# Autodesk Inventor assembly: CrossBot
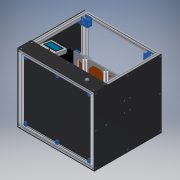
[picture p0: Inventor's stored thumbnail of the model, 180x180]
Saved by Autodesk Inventor 2016 (Build 200138000, 138)
## iProperties
Created: 2014-08-14
Part Number: CrossBot
Document SubType Name: Assembly
Designer: t_clevj
Mass: 16815.8 g
Surface Area: 53062.5 cm^2
Volume: 10946.1 cm^3
Density: 1.53623 g/cm^3
Author: t_clevj
## Documents named in this file (26)
- C:\Users\Jack\ownCloud\Projects\CrossBot\InventorModel\CrossBot.iam
- C:\Users\Jack\ownCloud\Projects\CrossBot\InventorModel\Frame\Frame.iam
- C:\Users\Jack\ownCloud\Projects\CrossBot\InventorModel\Hardware\Shaft\Shaft8\YShaft.ipt
- C:\Users\Jack\ownCloud\Projects\CrossBot\InventorModel\YAxis\YAxisMotorLeft.iam
- C:\Users\Jack\ownCloud\Projects\CrossBot\InventorModel\YAxis\YAxisIdlerLeft.iam
- C:\Users\Jack\ownCloud\Projects\CrossBot\InventorModel\YAxis\YAxisMotorRight.iam
- C:\Users\Jack\ownCloud\Projects\CrossBot\InventorModel\XAxis\XEndLeft.iam
- C:\Users\Jack\ownCloud\Projects\CrossBot\InventorModel\YAxis\YAxisIdlerRight.iam
- C:\Users\Jack\ownCloud\Projects\CrossBot\InventorModel\XAxis\XEndRight.iam
- C:\Users\Jack\ownCloud\Projects\CrossBot\InventorModel\Hardware\Shaft\Shaft8\XShaft.ipt
- C:\Users\Jack\ownCloud\Projects\CrossBot\InventorModel\Hardware\Shaft\Shaft10\ZAxisShaft.ipt
- C:\Users\Jack\ownCloud\Projects\CrossBot\InventorModel\Enclosure\SpoolFilamentToyBuilderLabs.ipt
- C:\Users\Jack\ownCloud\Projects\CrossBot\InventorModel\XAxis\XCarriage.iam
- C:\Users\Jack\ownCloud\Projects\CrossBot\InventorModel\Electronics\PSUUltibots.ipt
- C:\Users\Jack\ownCloud\Projects\CrossBot\InventorModel\ZAxis\ZAxisBed.iam
- C:\Users\Jack\ownCloud\Projects\CrossBot\InventorModel\ZAxis\ZAxisRodClamp.iam
- C:\Users\Jack\ownCloud\Projects\CrossBot\InventorModel\ZAxis\ZDrive.iam
- C:\Users\Jack\ownCloud\Projects\CrossBot\InventorModel\Electronics\KeySwitch\KeySwitch.iam
- C:\Users\Jack\ownCloud\Projects\CrossBot\InventorModel\ZAxis\ZEndstop.iam
- C:\Users\Jack\ownCloud\Projects\CrossBot\InventorModel\Electronics\Ports\PowerSocket.ipt
- C:\Users\Jack\ownCloud\Projects\CrossBot\InventorModel\Hardware\Nuts\ExtrusionNuts\ExtrusionNutHNKK5_4.ipt
- C:\Users\Jack\ownCloud\Projects\CrossBot\InventorModel\Electronics\Boards\RumbaBoard.ipt
- C:\Users\Jack\ownCloud\Projects\CrossBot\InventorModel\Enclosure\LCDCase\LCD+Case.iam
- C:\Users\Jack\ownCloud\Projects\CrossBot\InventorModel\Electronics\Boards\Raspi.ipt
- C:\Users\Jack\ownCloud\Projects\CrossBot\InventorModel\Extruder\ExtruderSatoer\ExtruderSatoerRight\ExtruderSatoerRight.iam
- C:\Users\Jack\ownCloud\Projects\CrossBot\InventorModel\Extruder\ExtruderSatoer\ExtruderSatoerLeft\ExtruderSatoerLeft.iam
## Components (61 placed, 25 different names)
1. Frame [sub-assembly] — Mate:6, Mate:23, Mate:24, Mate:25, Mate:27, Mate:28, Mate:29, Mate:30, Mate:31, Mate:32, Mate:69, Mate:70, Angle:13, Flush:92, Flush:93, Flush:94, Flush:95, Mate:352, Mate:353, Mate:354, Mate:355, Mate:381, Mate:382, Mate:383, Mate:400, Mate:401, Mate:402, Angle:46, Mate:417, Mate:418, Mate:419, Mate:426, Mate:427, Mate:428, Angle:47, Mate:465, Angle:50, Angle:51, Angle:52, Angle:53, Angle:54, Angle:55, Mate:466, Mate:467, Mate:468, Mate:469, Mate:470, Angle:56, Angle:58, Angle:59, Angle:60, Angle:61, Angle:62, Angle:63, Angle:64, Angle:65, Angle:66, Mate:471, Mate:472, Mate:473, Mate:474, Mate:475, Mate:476, Mate:477, Mate:478, Mate:479, Mate:480, Angle:67, Angle:68, Angle:69, Angle:70, Mate:481, Mate:482, Mate:483, Mate:484, Angle:71, Angle:72, Angle:73, Angle:74, Mate:485, Mate:486, Mate:487, Mate:488, Angle:75, Angle:76, Angle:77, Angle:78, Mate:489, Mate:490, Mate:491, Mate:492, Mate:497, Mate:498, Mate:517, Mate:518, Mate:519, Mate:520, Mate:521, Mate:522, Flush:98, Mate:526, Flush:99
2. ExtruderSatoerRight:1 [sub-assembly] — Mate:522, Mate:523, Mate:524, Flush:98, Mate:530
3. ExtruderSatoerLeft:1 [sub-assembly] — Mate:526, Mate:527, Mate:528, Flush:99, Mate:529
4. ZEndstop:1 [sub-assembly] — Mate:415, Angle:46, Mate:416
5. ZDrive:1 [sub-assembly] — Mate:381, Mate:382, Mate:383, Mate:384, Mate:431, Mate:459, Mate:460, Mate:461, Mate:462
6. ZAxisRodClamp:4 [sub-assembly] — Mate:350, Flush:95, Mate:355, Mate:384, Mate:455, Mate:456
7. ZAxisRodClamp:3 [sub-assembly] — Mate:349, Flush:94, Mate:352, Flush:97, Mate:416, Mate:463, Mate:464
8. ZAxisRodClamp:2 [sub-assembly] — Mate:348, Flush:92, Mate:354, Mate:457, Mate:458
9. ZAxisRodClamp:1 [sub-assembly] — Mate:347, Flush:93, Mate:353, Flush:96, Mate:449, Mate:450
10. ZAxisBed:1 [sub-assembly] — Mate:431, Angle:47
11. ZAxisShaft:1 — Mate:349, Mate:350, Mate:351, Flush:97, Mate:415
12. ZAxisShaft:2 — Mate:347, Mate:348, Mate:351, Flush:96
13. YShaft:2 — Mate:26, Mate:130, Mate:514
14. YShaft:3 — Mate:37, Mate:190
15. YAxisMotorLeft:1 [sub-assembly] — Mate:23, Mate:24, Mate:25, Mate:26, Mate:439, Mate:440, Mate:441, Mate:442, Mate:529
16. YAxisMotorRight:1 [sub-assembly] — Mate:30, Mate:31, Mate:32, Mate:37, Mate:435, Mate:436, Mate:437, Mate:438, Mate:530
17. YAxisIdlerLeft:1 [sub-assembly] — Mate:27, Mate:28, Mate:29, Mate:130, Mate:443, Mate:444, Mate:445
18. YAxisIdlerRight:1 [sub-assembly] — Mate:426, Mate:427, Mate:428, Mate:446, Mate:447, Mate:448
19. XShaft:1 — Mate:189, Flush:54, Mate:513, Mate:515
20. XShaft:2 — Mate:188, Flush:55, Mate:191, Mate:516
21. XCarriage:1 [sub-assembly] — Mate:515, Mate:516
22. XEndLeft:1 [sub-assembly] — Mate:188, Mate:189, Flush:54, Flush:55, Mate:514
23. XEndRight:1 [sub-assembly] — Mate:190, Mate:191, Angle:13, Mate:513
24. Raspi:1 — Mate:521
25. RumbaBoard:1 — Mate:498
26. LCD+Case:1 [sub-assembly]
27. KeySwitch:1 [sub-assembly] — Mate:400, Mate:401, Mate:402
28. PowerSocket:1 — Mate:417, Mate:418, Mate:419
29. PSUUltibots:1 — Mate:497
30. SpoolFilamentToyBuilderLabs:3 — Mate:517, Mate:518
31. SpoolFilamentToyBuilderLabs:4 — Mate:519, Mate:520
32. ExtrusionNutHNKK5_4:22 — Mate:455, Angle:51, Mate:469
33. ExtrusionNutHNKK5_4:30 — Mate:464, Angle:74, Mate:485
34. ExtrusionNutHNKK5_4:29 — Mate:463, Angle:71, Mate:486
35. ExtrusionNutHNKK5_4:16 — Mate:450, Angle:73, Mate:487
36. ExtrusionNutHNKK5_4:15 — Mate:449, Angle:72, Mate:488
37. ExtrusionNutHNKK5_4:23 — Mate:457, Angle:53, Mate:466
38. ExtrusionNutHNKK5_4:24 — Mate:458, Angle:54, Mate:470
39. ExtrusionNutHNKK5_4:21 — Mate:456, Mate:465, Angle:50
40. ExtrusionNutHNKK5_4:28 — Mate:462, Angle:55, Mate:468
41. ExtrusionNutHNKK5_4:27 — Mate:461, Angle:52, Mate:467
42. ExtrusionNutHNKK5_4:26 — Mate:459
43. ExtrusionNutHNKK5_4:25 — Mate:460
44. ExtrusionNutHNKK5_4:4 — Mate:438, Angle:76, Mate:492
45. ExtrusionNutHNKK5_4:1 — Mate:437, Angle:61, Mate:476
46. ExtrusionNutHNKK5_4:2 — Mate:436, Angle:63, Mate:474
47. ExtrusionNutHNKK5_4:3 — Mate:435, Angle:62, Mate:475
48. ExtrusionNutHNKK5_4:5 — Mate:442, Angle:75, Mate:491
49. ExtrusionNutHNKK5_4:6 — Mate:441, Angle:66, Mate:471
50. ExtrusionNutHNKK5_4:8 — Mate:439, Angle:64, Mate:473
51. ExtrusionNutHNKK5_4:7 — Mate:440, Angle:65, Mate:472
52. ExtrusionNutHNKK5_4:14 — Mate:448, Angle:78, Mate:489
53. ExtrusionNutHNKK5_4:12 — Mate:446, Angle:60, Mate:477
54. ExtrusionNutHNKK5_4:13 — Mate:447, Angle:56, Mate:478
55. ExtrusionNutHNKK5_4:10 — Mate:443, Angle:58, Mate:479
56. ExtrusionNutHNKK5_4:11 — Mate:445, Angle:59, Mate:480
57. ExtrusionNutHNKK5_4:9 — Mate:444, Angle:77, Mate:490
58. ExtrusionNutHNKK5_4:18 — Angle:67, Mate:483, Mate:524
59. ExtrusionNutHNKK5_4:17 — Angle:68, Mate:484, Mate:523
60. ExtrusionNutHNKK5_4:20 — Angle:69, Mate:481, Mate:527
61. ExtrusionNutHNKK5_4:19 — Angle:70, Mate:482, Mate:528
## Relationships (158: Mate 117, Angle 31, Flush 10)
- Mate:6: Frame
- Mate:23: Frame ↔ YAxisMotorLeft:1
- Mate:24: Frame ↔ YAxisMotorLeft:1
- Mate:25: Frame ↔ YAxisMotorLeft:1
- Mate:26: YShaft:2 ↔ YAxisMotorLeft:1
- Mate:27: Frame ↔ YAxisIdlerLeft:1
- Mate:28: Frame ↔ YAxisIdlerLeft:1
- Mate:29: Frame ↔ YAxisIdlerLeft:1
- Mate:30: Frame ↔ YAxisMotorRight:1
- Mate:31: Frame ↔ YAxisMotorRight:1
- Mate:32: Frame ↔ YAxisMotorRight:1
- Mate:37: YShaft:3 ↔ YAxisMotorRight:1
- Mate:69: Frame
- Mate:70: Frame
- Mate:130: YShaft:2 ↔ YAxisIdlerLeft:1
- Mate:188: XShaft:2 ↔ XEndLeft:1
- Mate:189: XShaft:1 ↔ XEndLeft:1
- Flush:54: XShaft:1 ↔ XEndLeft:1
- Flush:55: XShaft:2 ↔ XEndLeft:1
- Mate:190: YShaft:3 ↔ XEndRight:1
- Mate:191: XShaft:2 ↔ XEndRight:1
- Angle:13 (0 deg): Frame ↔ XEndRight:1
- Mate:347: ZAxisRodClamp:1 ↔ ZAxisShaft:2
- Mate:348: ZAxisRodClamp:2 ↔ ZAxisShaft:2
- Flush:92: Frame ↔ ZAxisRodClamp:2
- Flush:93: Frame ↔ ZAxisRodClamp:1
- Mate:349: ZAxisRodClamp:3 ↔ ZAxisShaft:1
- Flush:94: Frame ↔ ZAxisRodClamp:3
- Mate:350: ZAxisRodClamp:4 ↔ ZAxisShaft:1
- Flush:95: Frame ↔ ZAxisRodClamp:4
- Mate:351 (130 mm): ZAxisShaft:1 ↔ ZAxisShaft:2
- Mate:352: Frame ↔ ZAxisRodClamp:3
- Mate:353: Frame ↔ ZAxisRodClamp:1
- Mate:354: Frame ↔ ZAxisRodClamp:2
- Mate:355: Frame ↔ ZAxisRodClamp:4
- Flush:96: ZAxisRodClamp:1 ↔ ZAxisShaft:2
- Flush:97: ZAxisRodClamp:3 ↔ ZAxisShaft:1
- Mate:381: Frame ↔ ZDrive:1
- Mate:382: Frame ↔ ZDrive:1
- Mate:383 (187.5 mm): Frame ↔ ZDrive:1
- Mate:384 (24.5 mm): ZDrive:1 ↔ ZAxisRodClamp:4
- Mate:400: Frame ↔ KeySwitch:1
- Mate:401: Frame ↔ KeySwitch:1
- Mate:402: Frame ↔ KeySwitch:1
- Mate:415: ZEndstop:1 ↔ ZAxisShaft:1
- Angle:46 (0 deg): Frame ↔ ZEndstop:1
- Mate:416 (0.5 mm): ZEndstop:1 ↔ ZAxisRodClamp:3
- Mate:417: Frame ↔ PowerSocket:1
- Mate:418: Frame ↔ PowerSocket:1
- Mate:419: Frame ↔ PowerSocket:1
- Mate:426: Frame ↔ YAxisIdlerRight:1
- Mate:427: Frame ↔ YAxisIdlerRight:1
- Mate:428: Frame ↔ YAxisIdlerRight:1
- Mate:431: ZDrive:1 ↔ ZAxisBed:1
- Angle:47 (0 deg): Frame ↔ ZAxisBed:1
- Mate:435: YAxisMotorRight:1 ↔ ExtrusionNutHNKK5_4:3
- Mate:436: YAxisMotorRight:1 ↔ ExtrusionNutHNKK5_4:2
- Mate:437: YAxisMotorRight:1 ↔ ExtrusionNutHNKK5_4:1
- Mate:438: YAxisMotorRight:1 ↔ ExtrusionNutHNKK5_4:4
- Mate:439: YAxisMotorLeft:1 ↔ ExtrusionNutHNKK5_4:8
- Mate:440: YAxisMotorLeft:1 ↔ ExtrusionNutHNKK5_4:7
- Mate:441: YAxisMotorLeft:1 ↔ ExtrusionNutHNKK5_4:6
- Mate:442: YAxisMotorLeft:1 ↔ ExtrusionNutHNKK5_4:5
- Mate:443: YAxisIdlerLeft:1 ↔ ExtrusionNutHNKK5_4:10
- Mate:444: YAxisIdlerLeft:1 ↔ ExtrusionNutHNKK5_4:9
- Mate:445: YAxisIdlerLeft:1 ↔ ExtrusionNutHNKK5_4:11
- Mate:446: YAxisIdlerRight:1 ↔ ExtrusionNutHNKK5_4:12
- Mate:447: YAxisIdlerRight:1 ↔ ExtrusionNutHNKK5_4:13
- Mate:448: YAxisIdlerRight:1 ↔ ExtrusionNutHNKK5_4:14
- Mate:449: ZAxisRodClamp:1 ↔ ExtrusionNutHNKK5_4:15
- Mate:450: ZAxisRodClamp:1 ↔ ExtrusionNutHNKK5_4:16
- Mate:455: ZAxisRodClamp:4 ↔ ExtrusionNutHNKK5_4:22
- Mate:456: ZAxisRodClamp:4 ↔ ExtrusionNutHNKK5_4:21
- Mate:457: ZAxisRodClamp:2 ↔ ExtrusionNutHNKK5_4:23
- Mate:458: ZAxisRodClamp:2 ↔ ExtrusionNutHNKK5_4:24
- Mate:459: ZDrive:1 ↔ ExtrusionNutHNKK5_4:26
- Mate:460: ZDrive:1 ↔ ExtrusionNutHNKK5_4:25
- Mate:461: ZDrive:1 ↔ ExtrusionNutHNKK5_4:27
- Mate:462: ZDrive:1 ↔ ExtrusionNutHNKK5_4:28
- Mate:463: ZAxisRodClamp:3 ↔ ExtrusionNutHNKK5_4:29
- Mate:464: ZAxisRodClamp:3 ↔ ExtrusionNutHNKK5_4:30
- Mate:465: Frame ↔ ExtrusionNutHNKK5_4:21
- Angle:50 (0 deg): Frame ↔ ExtrusionNutHNKK5_4:21
- Angle:51 (0 deg): Frame ↔ ExtrusionNutHNKK5_4:22
- Angle:52 (0 deg): Frame ↔ ExtrusionNutHNKK5_4:27
- Angle:53 (0 deg): Frame ↔ ExtrusionNutHNKK5_4:23
- Angle:54 (0 deg): Frame ↔ ExtrusionNutHNKK5_4:24
- Angle:55 (0 deg): Frame ↔ ExtrusionNutHNKK5_4:28
- Mate:466: Frame ↔ ExtrusionNutHNKK5_4:23
- Mate:467: Frame ↔ ExtrusionNutHNKK5_4:27
- Mate:468: Frame ↔ ExtrusionNutHNKK5_4:28
- Mate:469: Frame ↔ ExtrusionNutHNKK5_4:22
- Mate:470: Frame ↔ ExtrusionNutHNKK5_4:24
- Angle:56 (0 deg): Frame ↔ ExtrusionNutHNKK5_4:13
- Angle:58 (0 deg): Frame ↔ ExtrusionNutHNKK5_4:10
- Angle:59 (0 deg): Frame ↔ ExtrusionNutHNKK5_4:11
- Angle:60 (0 deg): Frame ↔ ExtrusionNutHNKK5_4:12
- Angle:61 (0 deg): Frame ↔ ExtrusionNutHNKK5_4:1
- Angle:62 (0 deg): Frame ↔ ExtrusionNutHNKK5_4:3
- Angle:63 (0 deg): Frame ↔ ExtrusionNutHNKK5_4:2
- Angle:64 (0 deg): Frame ↔ ExtrusionNutHNKK5_4:8
- Angle:65 (0 deg): Frame ↔ ExtrusionNutHNKK5_4:7
- Angle:66 (0 deg): Frame ↔ ExtrusionNutHNKK5_4:6
- Mate:471: Frame ↔ ExtrusionNutHNKK5_4:6
- Mate:472: Frame ↔ ExtrusionNutHNKK5_4:7
- Mate:473: Frame ↔ ExtrusionNutHNKK5_4:8
- Mate:474: Frame ↔ ExtrusionNutHNKK5_4:2
- Mate:475: Frame ↔ ExtrusionNutHNKK5_4:3
- Mate:476: Frame ↔ ExtrusionNutHNKK5_4:1
- Mate:477: Frame ↔ ExtrusionNutHNKK5_4:12
- Mate:478: Frame ↔ ExtrusionNutHNKK5_4:13
- Mate:479: Frame ↔ ExtrusionNutHNKK5_4:10
- Mate:480: Frame ↔ ExtrusionNutHNKK5_4:11
- Angle:67 (0 deg): Frame ↔ ExtrusionNutHNKK5_4:18
- Angle:68 (0 deg): Frame ↔ ExtrusionNutHNKK5_4:17
- Angle:69 (0 deg): Frame ↔ ExtrusionNutHNKK5_4:20
- Angle:70 (0 deg): Frame ↔ ExtrusionNutHNKK5_4:19
- Mate:481: Frame ↔ ExtrusionNutHNKK5_4:20
- Mate:482: Frame ↔ ExtrusionNutHNKK5_4:19
- Mate:483: Frame ↔ ExtrusionNutHNKK5_4:18
- Mate:484: Frame ↔ ExtrusionNutHNKK5_4:17
- Angle:71 (0 deg): Frame ↔ ExtrusionNutHNKK5_4:29
- Angle:72 (0 deg): Frame ↔ ExtrusionNutHNKK5_4:15
- Angle:73 (0 deg): Frame ↔ ExtrusionNutHNKK5_4:16
- Angle:74 (0 deg): Frame ↔ ExtrusionNutHNKK5_4:30
- Mate:485: Frame ↔ ExtrusionNutHNKK5_4:30
- Mate:486: Frame ↔ ExtrusionNutHNKK5_4:29
- Mate:487: Frame ↔ ExtrusionNutHNKK5_4:16
- Mate:488: Frame ↔ ExtrusionNutHNKK5_4:15
- Angle:75 (0 deg): Frame ↔ ExtrusionNutHNKK5_4:5
- Angle:76 (0 deg): Frame ↔ ExtrusionNutHNKK5_4:4
- Angle:77 (0 deg): Frame ↔ ExtrusionNutHNKK5_4:9
- Angle:78 (0 deg): Frame ↔ ExtrusionNutHNKK5_4:14
- Mate:489: Frame ↔ ExtrusionNutHNKK5_4:14
- Mate:490: Frame ↔ ExtrusionNutHNKK5_4:9
- Mate:491: Frame ↔ ExtrusionNutHNKK5_4:5
- Mate:492: Frame ↔ ExtrusionNutHNKK5_4:4
- Mate:497: Frame ↔ PSUUltibots:1
- Mate:498: Frame ↔ RumbaBoard:1
- Mate:513: XShaft:1 ↔ XEndRight:1
- Mate:514: YShaft:2 ↔ XEndLeft:1
- Mate:515: XShaft:1 ↔ XCarriage:1
- Mate:516: XShaft:2 ↔ XCarriage:1
- Mate:517: Frame ↔ SpoolFilamentToyBuilderLabs:3
- Mate:518: Frame ↔ SpoolFilamentToyBuilderLabs:3
- Mate:519: Frame ↔ SpoolFilamentToyBuilderLabs:4
- Mate:520: Frame ↔ SpoolFilamentToyBuilderLabs:4
- Mate:521 (5 mm): Frame ↔ Raspi:1
- Mate:522: Frame ↔ ExtruderSatoerRight:1
- Mate:523: ExtruderSatoerRight:1 ↔ ExtrusionNutHNKK5_4:17
- Mate:524: ExtruderSatoerRight:1 ↔ ExtrusionNutHNKK5_4:18
- Flush:98: Frame ↔ ExtruderSatoerRight:1
- Mate:526: Frame ↔ ExtruderSatoerLeft:1
- Mate:527: ExtruderSatoerLeft:1 ↔ ExtrusionNutHNKK5_4:20
- Mate:528: ExtruderSatoerLeft:1 ↔ ExtrusionNutHNKK5_4:19
- Flush:99: Frame ↔ ExtruderSatoerLeft:1
- Mate:529 (12 mm): ExtruderSatoerLeft:1 ↔ YAxisMotorLeft:1
- Mate:530 (12 mm): ExtruderSatoerRight:1 ↔ YAxisMotorRight:1
